# Autodesk Inventor assembly: Wedge Dual Assembly
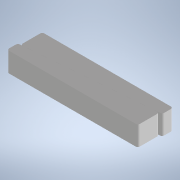
[picture p0: Inventor's stored thumbnail of the model, 180x180]
Saved by Autodesk Inventor 2020 (Build 240168000, 168)
## iProperties
Created: 2020-05-11
Part Number: Wedge Dual Assembly
Document SubType Name: Assembly
Designer: Dan Wikman
Author: Dan Wikman
## Documents named in this file (2)
- C:\Users\Dan Wikman\OneDrive\University Life\2020, Semester 1\METR4900 Honours Thesis\Full Scale Design\Wedge Dual Assembly.iam
- C:\Users\Dan Wikman\OneDrive\University Life\2020, Semester 1\METR4900 Honours Thesis\Full Scale Design\Wedge.ipt
## Components (2 placed, 1 different names)
1. Wedge:1 — Flush:1, Mate:1, Mate:2
2. Wedge:2 — Flush:1, Mate:1, Mate:2
## Relationships (3: Mate 2, Flush 1)
- Flush:1: Wedge:1 ↔ Wedge:2
- Mate:1: Wedge:1 ↔ Wedge:2
- Mate:2 (-30 mm): Wedge:1 ↔ Wedge:2
